# Autodesk Inventor assembly: am-3480 4IN 500Hex Compliant Wheel REV2
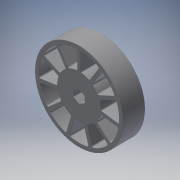
[picture p0: Inventor's stored thumbnail of the model, 180x180]
Saved by Autodesk Inventor 2017 (Build 210142000, 142)
## iProperties
Created: 2019-10-29
Part Number: am-3480 4IN 500Hex Compliant Wheel REV2
Description: STEP AP203
Document SubType Name: Assembly
Designer: S347110131
Sending System: SolidWorks 2019
Preprocessor: SwSTEP 2.0
Title: am-3480 4IN 500Hex Bore Compliant Wheel REV2.STEP
Revision Number: ANY
## Documents named in this file (3)
- P:\Robotics\2020 INFINIT RECHARGE\Panel\New_Spinning_Idea\am-3480 4IN 500Hex Compliant Wheel REV2.iam
- P:\Robotics\2020 INFINIT RECHARGE\Panel\New_Spinning_Idea\4IN Compliant Wheel FINAL Overmold.ipt
- P:\Robotics\2020 INFINIT RECHARGE\Panel\New_Spinning_Idea\2in Wheel Intergrated 0500 HEX Hub.ipt
## Components (2 placed, 2 different names)
1. 4IN Compliant Wheel FINAL Overmold_1 — Mate:1, Mate:2
2. 2in Wheel Intergrated 0500 HEX Hub_2 — Mate:1, Mate:2
## Relationships (2: Mate 2)
- Mate:1: 4IN Compliant Wheel FINAL Overmold_1 ↔ 2in Wheel Intergrated 0500 HEX Hub_2
- Mate:2: 4IN Compliant Wheel FINAL Overmold_1 ↔ 2in Wheel Intergrated 0500 HEX Hub_2
